# Autodesk Inventor assembly: XY Drive Subassy
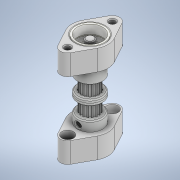
[picture p0: Inventor's stored thumbnail of the model, 180x180]
Saved by Autodesk Inventor 2022 (Build 260153000, 153)
## iProperties
Created: 2021-10-06
Part Number: XY Drive Subassy
Document SubType Name: Assembly
Designer: nicol
Author: nicol
## Documents named in this file (6)
- C:\Users\nicol\Documents\_Origami Printer\XY Drive Subassy.iam
- C:\Users\nicol\Documents\_Origami Printer\Bearings\625 Bearing.ipt
- C:\Users\nicol\Documents\_Origami Printer\3D printed\XY Drive Bearing Holder.ipt
- C:\Users\nicol\Documents\_Origami Printer\Hardware\GT2 Pulley 16T.ipt
- C:\Users\nicol\Documents\_Origami Printer\Hardware\5 x 50mm Shaft.ipt
- C:\Users\nicol\Documents\_Origami Printer\3D printed\Bearing Retaining Ring.ipt
## Components (9 placed, 5 different names)
1. 625 Bearing:1 — Insert:2, Insert:5, Insert:6, Insert:7
2. 625 Bearing:2 — Insert:1, Insert:3, Insert:8
3. XY Drive Bearing Holder:1 — Insert:1
4. XY Drive Bearing Holder:2 — Insert:2
5. GT2 Pulley 16T:1 — Insert:4, Insert:5
6. GT2 Pulley 16T:2 — Insert:3, Insert:4
7. 5 x 50mm Shaft:1 — Insert:6
8. Bearing Retaining Ring:1 — Insert:7
9. Bearing Retaining Ring:2 — Insert:8
## Relationships (8: Insert 8)
- Insert:1: 625 Bearing:2 ↔ XY Drive Bearing Holder:1
- Insert:2: 625 Bearing:1 ↔ XY Drive Bearing Holder:2
- Insert:3 (3 mm): 625 Bearing:2 ↔ GT2 Pulley 16T:2
- Insert:4: GT2 Pulley 16T:1 ↔ GT2 Pulley 16T:2
- Insert:5: 625 Bearing:1 ↔ GT2 Pulley 16T:1
- Insert:6 (-3 mm): 625 Bearing:1 ↔ 5 x 50mm Shaft:1
- Insert:7: 625 Bearing:1 ↔ Bearing Retaining Ring:1
- Insert:8: 625 Bearing:2 ↔ Bearing Retaining Ring:2
